# Autodesk Inventor assembly: box example
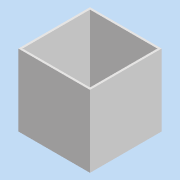
[picture p0: Inventor's stored thumbnail of the model, 180x180]
Saved by Autodesk Inventor 2020 (Build 240168000, 168)
## iProperties
Created: 2020-12-17
Part Number: box example
Document SubType Name: Assembly
Designer: solar
Author: solar
## Documents named in this file (2)
- D:\S.olar\College stuff\3 Junior\Term 5\MCT 131 Introductions to Mechatronics\FINAL INVENTOR\box\box example.iam
- D:\S.olar\College stuff\3 Junior\Term 5\MCT 131 Introductions to Mechatronics\FINAL INVENTOR\box\simple wall test.ipt
## Components (4 placed, 1 different names)
1. simple wall test:1 — Mate:3, Angle:2, Mate:4, Mate:7
2. simple wall test:2 — Mate:1, Angle:1, Mate:2, Mate:3, Angle:2, Mate:4
3. simple wall test:3 — Mate:6, Angle:3, Mate:7
4. simple wall test:4 — Mate:1, Angle:1, Mate:2, Mate:6, Angle:3
## Relationships (9: Mate 6, Angle 3)
- Mate:1: simple wall test:2 ↔ simple wall test:4
- Angle:1 (90 deg): simple wall test:2 ↔ simple wall test:4
- Mate:2: simple wall test:2 ↔ simple wall test:4
- Mate:3: simple wall test:1 ↔ simple wall test:2
- Angle:2 (270 deg): simple wall test:1 ↔ simple wall test:2
- Mate:4: simple wall test:1 ↔ simple wall test:2
- Mate:6: simple wall test:3 ↔ simple wall test:4
- Angle:3 (90 deg): simple wall test:3 ↔ simple wall test:4
- Mate:7: simple wall test:1 ↔ simple wall test:3
